# Autodesk Inventor assembly: !tower
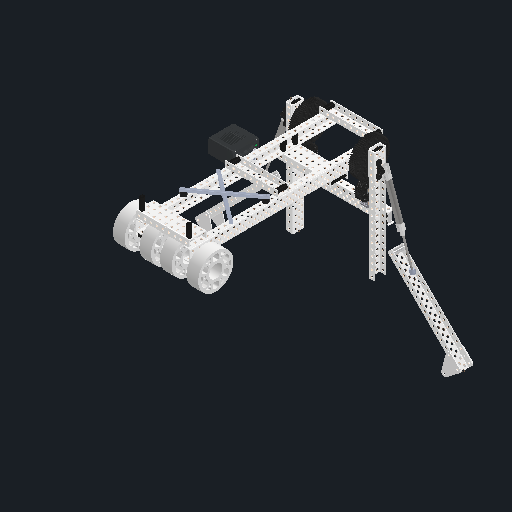
[picture p0: Inventor's stored thumbnail of the model, 512x512]
Saved by Autodesk Inventor 2024 (Build 280153000, 153)
## iProperties
Created: 2024-01-16
Part Number: !tower
Document SubType Name: Assembly
Designer: Averey Ku
Author: Averey Ku
## Documents named in this file (9)
- C:\Users\avere\Documents\rbp_cad\zoomba_v0.3\tower\!tower.iam
- C:\Users\avere\Documents\rbp_cad\zoomba_v0.3\tower\side.iam
- C:\Users\avere\Documents\rbp_cad\zoomba_v0.3\tower\mirrored_parts\tower_MIR.iam
- C:\Users\avere\Documents\rbp_cad\VEX-CAD-Inventor-1.41\Structure\C Channel\Aluminum 1x2x1\Alu C 1x2x1x15.ipt
- C:\Users\avere\Documents\rbp_cad\hardware\.375 OD Aluminum Spacer 0.875.ipt
- C:\Users\avere\Documents\rbp_cad\zoomba_v0.3\arm\!arm.iam
- C:\Users\avere\Documents\rbp_cad\VEX-CAD-Inventor-1.41\Motion\Gears\HS Gear\HS 36T Gear, No Insert.iam
- C:\Users\avere\Documents\rbp_cad\VEX-CAD-Inventor-1.41\Motion\Gears\HS Gear.iam
- C:\Users\avere\Documents\rbp_cad\VEX-CAD-Inventor-1.41\Motion\Gears\HS Gear\HS 12T Gear, No Insert.iam
## Components (9 placed, 7 different names)
1. side:1 [sub-assembly] — Insert:1, Mate:1, Insert:5, Insert:6, Insert:8
2. tower_MIR:1 [sub-assembly] — Insert:2, Mate:2, Insert:7
3. Alu C 1x2x1x15:1 — Insert:1, Mate:1, Insert:2, Mate:2, Insert:3, Insert:4
4. .375 OD Aluminum Spacer 0.875:1 — Insert:4
5. .375 OD Aluminum Spacer 0.875:2 — Insert:3
6. !arm:1 [sub-assembly] — Insert:5
7. HS 36T Gear, No Insert:1 [sub-assembly] — Insert:6
8. HS 36T Gear, No Insert:2 [sub-assembly] — Insert:7
9. HS 12T Gear, No Insert:3 [sub-assembly] — Insert:8
## Relationships (10: Insert 8, Mate 2)
- Insert:1: side:1 ↔ Alu C 1x2x1x15:1
- Mate:1: side:1 ↔ Alu C 1x2x1x15:1
- Insert:2: tower_MIR:1 ↔ Alu C 1x2x1x15:1
- Mate:2: tower_MIR:1 ↔ Alu C 1x2x1x15:1
- Insert:3: Alu C 1x2x1x15:1 ↔ .375 OD Aluminum Spacer 0.875:2
- Insert:4: Alu C 1x2x1x15:1 ↔ .375 OD Aluminum Spacer 0.875:1
- Insert:5 (9.525 mm): side:1 ↔ !arm:1
- Insert:6 (9.525 mm): side:1 ↔ HS 36T Gear, No Insert:1
- Insert:7 (9.525 mm): tower_MIR:1 ↔ HS 36T Gear, No Insert:2
- Insert:8 (9.525 mm): side:1 ↔ HS 12T Gear, No Insert:3
